# Autodesk Inventor assembly: BaseEnsamble
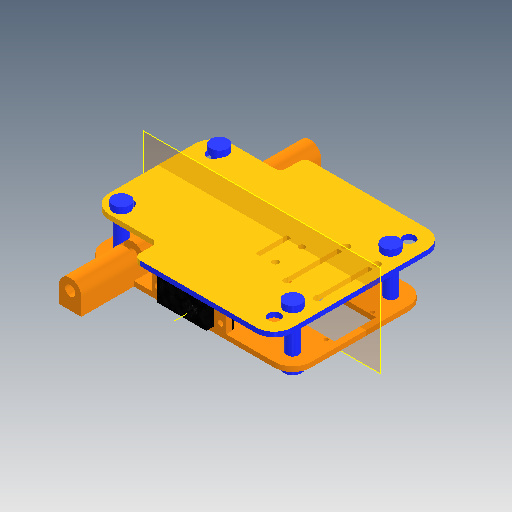
[picture p0: Inventor's stored thumbnail of the model, 512x512]
Saved by Autodesk Inventor 2021 (Build 250183000, 183)
## iProperties
Created: 2024-04-08
Part Number: BaseEnsamble
Document SubType Name: Assembly
Designer: Martin
Mass: 327.621 g
Surface Area: 1126.86 cm^2
Volume: 257.969 cm^3
Density: 1.27 g/cm^3
Author: Martin
## Documents named in this file (6)
- C:\Users\ASUS\OneDrive - Universidad de Antioquia\2024-1\Robótica\Proyecto\CAD\op1\BaseEnsamble.iam
- C:\Users\ASUS\OneDrive - Universidad de Antioquia\2024-1\Robótica\Proyecto\CAD\op1\Base.ipt
- C:\Users\ASUS\OneDrive - Universidad de Antioquia\2024-1\Robótica\Proyecto\CAD\op1\Base2.ipt
- C:\Users\ASUS\OneDrive - Universidad de Antioquia\2024-1\Robótica\Proyecto\CAD\op1\PasadorBase.ipt
- C:\Users\ASUS\OneDrive - Universidad de Antioquia\2024-1\Robótica\Proyecto\CAD\op1\TapaPasador.ipt
- C:\Users\ASUS\OneDrive - Universidad de Antioquia\2024-1\Robótica\Proyecto\CAD\Servo.ipt
## Components (13 placed, 5 different names)
1. Base:1 — Mate:9, Mate:10, Mate:11, Mate:17, Mate:18, Mate:19, Mate:20, Mate:21, Mate:22, Mate:24, Mate:26, Mate:27
2. Base2:1 — Mate:1, Mate:2, Mate:3, Mate:4, Mate:5, Mate:6, Mate:7, Mate:8, Mate:9
3. PasadorBase:1 — Mate:1, Mate:5, Mate:11, Mate:14
4. PasadorBase:2 — Mate:2, Mate:6, Mate:13
5. PasadorBase:3 — Mate:3, Mate:7, Mate:10, Mate:16
6. PasadorBase:4 — Mate:4, Mate:8, Mate:15, Mate:28
7. TapaPasador:1 — Mate:15, Mate:18
8. TapaPasador:2 — Mate:16
9. TapaPasador:3 — Mate:13, Mate:17
10. TapaPasador:4 — Mate:14, Mate:19
11. Servo:1 — Mate:20, Mate:21, Mate:22
12. Servo:3 — Mate:24, Mate:26
13. TapaPasador:5 — Mate:27, Mate:28
## Relationships (26: Mate 25, Flush 1)
- Mate:1: Base2:1 ↔ PasadorBase:1
- Mate:2: Base2:1 ↔ PasadorBase:2
- Mate:3: Base2:1 ↔ PasadorBase:3
- Mate:4: Base2:1 ↔ PasadorBase:4
- Mate:5: Base2:1 ↔ PasadorBase:1
- Mate:6: Base2:1 ↔ PasadorBase:2
- Mate:7: Base2:1 ↔ PasadorBase:3
- Mate:8: Base2:1 ↔ PasadorBase:4
- Mate:9 (28 mm): Base:1 ↔ Base2:1
- Mate:10: Base:1 ↔ PasadorBase:3
- Mate:11: Base:1 ↔ PasadorBase:1
- Mate:13: PasadorBase:2 ↔ TapaPasador:3
- Mate:14: PasadorBase:1 ↔ TapaPasador:4
- Mate:15: PasadorBase:4 ↔ TapaPasador:1
- Mate:16: PasadorBase:3 ↔ TapaPasador:2
- Mate:17: Base:1 ↔ TapaPasador:3
- Mate:18: Base:1 ↔ TapaPasador:1
- Mate:19: Base:1 ↔ TapaPasador:4
- Mate:20: Base:1 ↔ Servo:1
- Mate:21: Base:1 ↔ Servo:1
- Mate:22 (64 mm): Base:1 ↔ Servo:1
- Mate:24: Base:1 ↔ Servo:3
- Mate:26: Base:1 ↔ Servo:3
- Flush:3 (-55 mm)
- Mate:27: Base:1 ↔ TapaPasador:5
- Mate:28: PasadorBase:4 ↔ TapaPasador:5
